# Autodesk Inventor assembly: MaquinaDeCorte
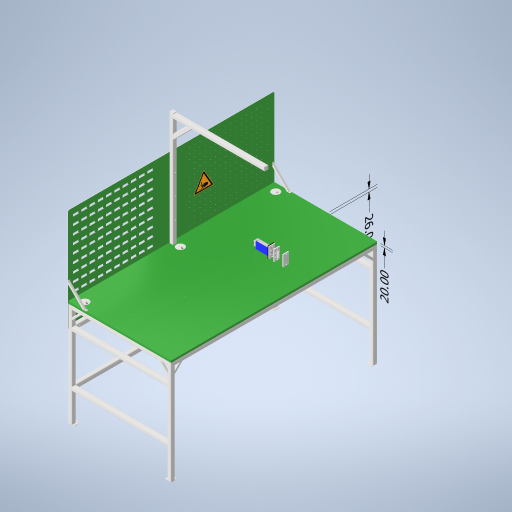
[picture p0: Inventor's stored thumbnail of the model, 512x512]
Saved by Autodesk Inventor 2023 (Build 270158000, 158)
## iProperties
Created: 2023-04-07
Part Number: MaquinaDeCorte
Document SubType Name: Assembly
Designer: Lenovo
Author: Lenovo
## Documents named in this file (13)
- D:\Esdek\Gemelo Digital\Corte de Tubos\MaquinaDeCorte.iam
- D:\Esdek\Gemelo Digital\Corte de Tubos\CADimportados\PistónElectromecánico\1470706 EPCO-25-300-3P-ST-E---(0).iam
- D:\Esdek\Gemelo Digital\Corte de Tubos\SoporteElectromecánico.ipt
- D:\Esdek\Gemelo Digital\Corte de Tubos\CADimportados\Main Table Assembly.ipt
- D:\Esdek\Gemelo Digital\Corte de Tubos\CADimportados\PistónHidráulico\163321 DNC-32-50-PPV---(asm_0).iam
- D:\Esdek\Gemelo Digital\Corte de Tubos\SoporteHidráhulicos.ipt
- D:\Esdek\Gemelo Digital\Corte de Tubos\PlacaSuperiorHidráulicos.ipt
- D:\Esdek\Gemelo Digital\Corte de Tubos\CodoHidráulicos.ipt
- D:\Esdek\Gemelo Digital\Corte de Tubos\PlacaMediaHidráulicos.ipt
- D:\Esdek\Gemelo Digital\Corte de Tubos\Cuchilla.ipt
- D:\Esdek\Gemelo Digital\Corte de Tubos\PlacaBaseHidráulicos.ipt
- D:\Esdek\Gemelo Digital\Corte de Tubos\BaseCuchilla.ipt
- D:\Esdek\Gemelo Digital\Corte de Tubos\CADimportados\Knutec.de - Warning, Crushing of hands, according ISO EN DIN 7010_200.ipt
## Components (12 placed, 12 different names)
1. 1470706 EPCO-25-300-3P-ST-E---(0):1 [sub-assembly] — Mate:30, Mate:31, Mate:32
2. Main Table Assembly:1 — Mate:25, Angle:1, Mate:26, Mate:27, Mate:28, Mate:29
3. 163321 DNC-32-50-PPV---(asm_0):1 [sub-assembly] — Mate:4, Mate:5, Mate:6, Mate:12
4. SoporteHidráhulicos:1 — Mate:4, Mate:5, Mate:6, Mate:7, Mate:8, Mate:9
5. PlacaSuperiorHidráulicos:1 — Mate:7, Mate:8, Mate:9, Mate:10, Mate:11, Mate:24
6. CodoHidráulicos:1 — Mate:10, Mate:11, Mate:12, Mate:13, Mate:14, Mate:15
7. PlacaMediaHidráulicos:1 — Mate:13, Mate:14, Mate:15, Mate:16, Mate:17, Mate:18, Mate:22, Mate:23
8. Cuchilla:1 — Mate:16, Mate:17, Mate:18
9. PlacaBaseHidráulicos:1 — Mate:19, Mate:20, Mate:21, Mate:22, Mate:23
10. BaseCuchilla:1 — Mate:19, Mate:20, Mate:21, Mate:24
11. Knutec.de - Warning, Crushing of hands, according ISO EN DIN 7010_200:1 — Mate:25, Angle:1, Mate:26
12. SoporteElectromecánico:1 — Mate:27, Mate:28, Mate:29, Mate:30, Mate:31, Mate:32
## Relationships (30: Mate 29, Angle 1)
- Mate:4: 163321 DNC-32-50-PPV---(asm_0):1 ↔ SoporteHidráhulicos:1
- Mate:5: 163321 DNC-32-50-PPV---(asm_0):1 ↔ SoporteHidráhulicos:1
- Mate:6: 163321 DNC-32-50-PPV---(asm_0):1 ↔ SoporteHidráhulicos:1
- Mate:7: SoporteHidráhulicos:1 ↔ PlacaSuperiorHidráulicos:1
- Mate:8: SoporteHidráhulicos:1 ↔ PlacaSuperiorHidráulicos:1
- Mate:9: SoporteHidráhulicos:1 ↔ PlacaSuperiorHidráulicos:1
- Mate:10: PlacaSuperiorHidráulicos:1 ↔ CodoHidráulicos:1
- Mate:11: PlacaSuperiorHidráulicos:1 ↔ CodoHidráulicos:1
- Mate:12: 163321 DNC-32-50-PPV---(asm_0):1 ↔ CodoHidráulicos:1
- Mate:13: CodoHidráulicos:1 ↔ PlacaMediaHidráulicos:1
- Mate:14: CodoHidráulicos:1 ↔ PlacaMediaHidráulicos:1
- Mate:15: CodoHidráulicos:1 ↔ PlacaMediaHidráulicos:1
- Mate:16: PlacaMediaHidráulicos:1 ↔ Cuchilla:1
- Mate:17: PlacaMediaHidráulicos:1 ↔ Cuchilla:1
- Mate:18: PlacaMediaHidráulicos:1 ↔ Cuchilla:1
- Mate:19: PlacaBaseHidráulicos:1 ↔ BaseCuchilla:1
- Mate:20: PlacaBaseHidráulicos:1 ↔ BaseCuchilla:1
- Mate:21: PlacaBaseHidráulicos:1 ↔ BaseCuchilla:1
- Mate:22: PlacaMediaHidráulicos:1 ↔ PlacaBaseHidráulicos:1
- Mate:23: PlacaMediaHidráulicos:1 ↔ PlacaBaseHidráulicos:1
- Mate:24 (115.5 mm): PlacaSuperiorHidráulicos:1 ↔ BaseCuchilla:1
- Mate:25: Main Table Assembly:1 ↔ Knutec.de - Warning, Crushing of hands, according ISO EN DIN 7010_200:1
- Angle:1 (180 deg): Main Table Assembly:1 ↔ Knutec.de - Warning, Crushing of hands, according ISO EN DIN 7010_200:1
- Mate:26: Main Table Assembly:1 ↔ Knutec.de - Warning, Crushing of hands, according ISO EN DIN 7010_200:1
- Mate:27: Main Table Assembly:1 ↔ SoporteElectromecánico:1
- Mate:28: Main Table Assembly:1 ↔ SoporteElectromecánico:1
- Mate:29: Main Table Assembly:1 ↔ SoporteElectromecánico:1
- Mate:30: 1470706 EPCO-25-300-3P-ST-E---(0):1 ↔ SoporteElectromecánico:1
- Mate:31: 1470706 EPCO-25-300-3P-ST-E---(0):1 ↔ SoporteElectromecánico:1
- Mate:32: 1470706 EPCO-25-300-3P-ST-E---(0):1 ↔ SoporteElectromecánico:1
